# Autodesk Inventor assembly: ASM2
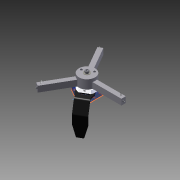
[picture p0: Inventor's stored thumbnail of the model, 180x180]
Saved by Autodesk Inventor 2011 SP2 (Build 150309200, 309)
## iProperties
Created: 2013-02-08
Part Number: ASM2
Document SubType Name: Assembly
Designer: sungwook
Author: sungwook
## Documents named in this file (11)
- C:\Users\sungwook\Documents\Inventor\Micron22_top_adj_02082013\02082012_Fiducail_Markers\ASM2.iam
- C:\Users\sungwook\Documents\Inventor\Micron22_top_adj_02082013\Parts\Tool\Tool Mount_Rev.ipt
- C:\Users\sungwook\Documents\Inventor\Micron22_top_adj_02082013\02082012_Fiducail_Markers\Fiducial_Post.ipt
- C:\Users\sungwook\Documents\Inventor\Micron22_top_adj_02082013\Parts\Main\Platform_Top_14mm_Rev.ipt
- C:\Users\sungwook\Documents\Inventor\Micron22_top_adj_02082013\02082012_Fiducail_Markers\Short_Needle.ipt
- C:\Users\sungwook\Documents\Inventor\Content Center Files\R2011\en-US\ANSI B18.3(18)\ANSI B18.3 - 0-80 UNF - 0.13(28).ipt
- C:\Users\sungwook\Documents\Inventor\Micron22_top_adj_02082013\Parts\ASAP\ASAP_Top_Fixture_New.ipt
- C:\Users\sungwook\Documents\Inventor\Content Center Files\R2011\en-US\ANSI B18.3(05)\ANSI B18.3 - 0-80 UNF - 1(31).ipt
- C:\Users\sungwook\Documents\Inventor\Micron22_top_adj_02082013\Imported Components\90107A001\washer_0.ipt
- C:\Users\sungwook\Documents\Inventor\Content Center Files\R2011\en-US\ANSI B18.3(13)\ANSI B18.3 - 0-80 UNF - 0.5(22).ipt
- C:\Users\sungwook\Documents\Inventor\Content Center Files\R2011\en-US\ANSI B18.6.3(36)\ANSI B18.6.3 - 0 - 80(2).ipt
## Components (15 placed, 10 different names)
1. Platform_Top_14mm_Rev:1 — Mate:9, Mate:10, Mate:11, Mate:19, Mate:20, Mate:21
2. Tool Mount_Rev:1 — Mate:9, Mate:10, Mate:11, Mate:15, Mate:16, Mate:22, Mate:23, Mate:27
3. Fiducial_Post:1 — Mate:12, Mate:13, Mate:14, Flush:1, Mate:15, Mate:16, Mate:22, Mate:23, Mate:24, Mate:25, Mate:26, Mate:28, Mate:29, Insert:1
4. ASAP_Top_Fixture_New:1 — Mate:19, Mate:20, Mate:21
5. Hexagon Socket Head Cap Screw - Inch 0-80 UNF - 1:1 — Mate:24, Mate:25
6. washer_0:1 — Mate:26, Mate:27, Flush:31
7. washer_0:2 — Mate:28, Mate:29
8. Spline Socket Head Cap Screw - Inch 0-80 UNF - 0.5:1 — Insert:1, Mate:30
9. Hex Machine Screw Nut - Inch 0 - 80:1 — Mate:30, Flush:31
10. Short_Needle:1 — Mate:12, Mate:13
11. Type A - Hexagon Socket Set Screw - Cup Point - Inch 0-80 UNF x 0.13:1 — Mate:14, Flush:1
12. Short_Needle:2
13. Type A - Hexagon Socket Set Screw - Cup Point - Inch 0-80 UNF x 0.13:2
14. Short_Needle:3
15. Type A - Hexagon Socket Set Screw - Cup Point - Inch 0-80 UNF x 0.13:3
## Component patterns: (3 elements, first: Short_Needle:1 + Type A - Hexagon Socket Set Screw - Cup Point - Inch 0-80 UNF x 0.13:1)
## Relationships (23: Mate 20, Flush 2, Insert 1)
- Mate:9: Platform_Top_14mm_Rev:1 ↔ Tool Mount_Rev:1
- Mate:10: Platform_Top_14mm_Rev:1 ↔ Tool Mount_Rev:1
- Mate:11: Platform_Top_14mm_Rev:1 ↔ Tool Mount_Rev:1
- Mate:12: Fiducial_Post:1 ↔ Short_Needle:1
- Mate:13: Fiducial_Post:1 ↔ Short_Needle:1
- Flush:1 (-0.5 mm): Fiducial_Post:1 ↔ Type A - Hexagon Socket Set Screw - Cup Point - Inch 0-80 UNF x 0.13:1
- Mate:15: Tool Mount_Rev:1 ↔ Fiducial_Post:1
- Mate:16: Tool Mount_Rev:1 ↔ Fiducial_Post:1
- Mate:19: Platform_Top_14mm_Rev:1 ↔ ASAP_Top_Fixture_New:1
- Mate:20: Platform_Top_14mm_Rev:1 ↔ ASAP_Top_Fixture_New:1
- Mate:21: Platform_Top_14mm_Rev:1 ↔ ASAP_Top_Fixture_New:1
- Mate:22: Tool Mount_Rev:1 ↔ Fiducial_Post:1
- Mate:23: Tool Mount_Rev:1 ↔ Fiducial_Post:1
- Mate:25: Fiducial_Post:1 ↔ Hexagon Socket Head Cap Screw - Inch 0-80 UNF - 1:1
- Mate:26: Fiducial_Post:1 ↔ washer_0:1
- Mate:27: Tool Mount_Rev:1 ↔ washer_0:1
- Mate:28: Fiducial_Post:1 ↔ washer_0:2
- Mate:29: Fiducial_Post:1 ↔ washer_0:2
- Flush:31: washer_0:1 ↔ Hex Machine Screw Nut - Inch 0 - 80:1
- Mate:14: Fiducial_Post:1 ↔ Type A - Hexagon Socket Set Screw - Cup Point - Inch 0-80 UNF x 0.13:1
- Mate:24: Fiducial_Post:1 ↔ Hexagon Socket Head Cap Screw - Inch 0-80 UNF - 1:1
- Insert:1: Fiducial_Post:1 ↔ Spline Socket Head Cap Screw - Inch 0-80 UNF - 0.5:1
- Mate:30: Spline Socket Head Cap Screw - Inch 0-80 UNF - 0.5:1 ↔ Hex Machine Screw Nut - Inch 0 - 80:1
